# Autodesk Inventor assembly: hand_motor_setter_base_under_assy
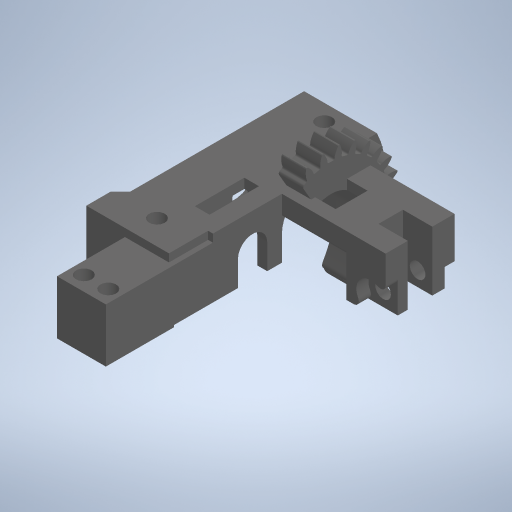
[picture p0: Inventor's stored thumbnail of the model, 512x512]
Saved by Autodesk Inventor 2024.1 (Build 281209000, 209)
## iProperties
Created: 2025-03-02
Part Number: hand_motor_setter_base_under_assy
Document SubType Name: Assembly
Designer: hibik
Author: hibik
## Documents named in this file (3)
- C:\Users\hibik\Documents\Robomech\RESCUE\ORCA\hard\arm\hand_motor_setter_base_under_assy.iam
- C:\Users\hibik\Documents\Robomech\RESCUE\ORCA\hard\arm\hand_gear_hand.ipt
- C:\Users\hibik\Documents\Robomech\RESCUE\ORCA\hard\arm\hand_motor_setter_base_under.ipt
## Components (2 placed, 2 different names)
1. hand_motor_setter_base_under:1 — 挿入:1, 角度:1
2. hand_gear_hand:1 — 挿入:1, 角度:1
## Relationships (2: Insert 1, Angle 1)
- 挿入:1 [Insert] (6 mm): hand_motor_setter_base_under:1 ↔ hand_gear_hand:1
- 角度:1 [Angle] (30 deg): hand_motor_setter_base_under:1 ↔ hand_gear_hand:1
